# Autodesk Inventor assembly: Quadropod_assembly_v3
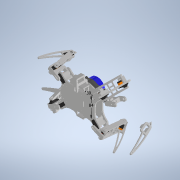
[picture p0: Inventor's stored thumbnail of the model, 180x180]
Saved by Autodesk Inventor 2020.3 (Build 243373000, 373)
## iProperties
Created: 2021-04-02
Part Number: Quadropod_assembly_v3
Document SubType Name: Assembly
Designer: sanyi
Author: sanyi
## Documents named in this file (14)
- C:\Users\sanyi\Documents\Inventor\Quadropod\Quadropod_assembly_v3.iam
- C:\Users\sanyi\Documents\Inventor\Quadropod\BaseBottom_v1.ipt
- C:\Users\sanyi\Documents\Inventor\Quadropod\BaseTop_v1.ipt
- C:\Users\sanyi\Documents\Inventor\Quadropod\LegPin_Middle_v1.ipt
- C:\Users\sanyi\Documents\Inventor\Quadropod\LegPin_Side_v1.ipt
- C:\Users\sanyi\Documents\Inventor\Quadropod\LegPin_Side_v1_MIR.ipt
- C:\Users\sanyi\Documents\Inventor\Quadropod\LegStart_v1.ipt
- C:\Users\sanyi\Documents\Inventor\Quadropod\LegEnd_Right_v2.ipt
- C:\Users\sanyi\Documents\Inventor\Quadropod\LegMiddle_Final_1.ipt
- C:\Users\sanyi\Documents\Inventor\Quadropod\LegPin_v1.ipt
- C:\Users\sanyi\Documents\Inventor\Quadropod\SH-0257MG.ipt
- C:\Users\sanyi\Documents\Inventor\Quadropod\ydlidar x4.ipt
- C:\Users\sanyi\Documents\Inventor\Quadropod\LegEnd_Right_v2_MIR.ipt
- C:\Users\sanyi\Documents\Inventor\Quadropod\LegStart_v1_MIR1.ipt
## Components (44 placed, 13 different names)
1. BaseBottom_v1:1 — Mate:1, Mate:2, Insert:15, Angle:1, Insert:31, Insert:32, Insert:34, Insert:35, Insert:36, Insert:37, Insert:38, Insert:39, Insert:40, Insert:41, Insert:42, Insert:43, Insert:72, Angle:10, Insert:73, Angle:11, Insert:74, Angle:12, Flush:4
2. BaseTop_v1:1 — Insert:75, Insert:76, Insert:77, Insert:78
3. LegPin_Side_v1:1 — Insert:42, Insert:43, Insert:79
4. LegPin_Side_v1_MIR:1 — Insert:40, Insert:41
5. LegPin_Middle_v1:5 — Insert:31, Insert:32, Insert:75
6. LegPin_Middle_v1:2 — Insert:36, Insert:37
7. LegPin_Middle_v1:3 — Insert:38, Insert:39, Insert:76
8. LegPin_Middle_v1:4 — Insert:34, Insert:35
9. LegStart_v1:1 — Insert:16, Insert:17, Angle:2, Flush:2, Insert:29, Insert:30
10. LegEnd_Right_v2:1 — Insert:23, Angle:3, Flush:3, Insert:27, Insert:28
11. LegMiddle_Final_1:1 — Insert:18, Insert:24
12. LegPin_v1:1 — Insert:29, Insert:30
13. LegPin_v1:2 — Insert:27, Insert:28
14. SH-0257MG:1 — Insert:15, Angle:1, Insert:16
15. SH-0257MG:2 — Insert:17, Angle:2, Insert:18
16. SH-0257MG:3 — Insert:23, Angle:3, Insert:24
17. LegStart_v1:2
18. LegEnd_Right_v2:2
19. LegMiddle_Final_1:2
20. LegPin_v1:3
21. LegPin_v1:4
22. SH-0257MG:4 — Insert:72, Angle:10
23. SH-0257MG:5
24. SH-0257MG:6
25. LegStart_v1:3
26. LegEnd_Right_v2:3
27. LegMiddle_Final_1:3
28. LegPin_v1:5
29. LegPin_v1:6
30. SH-0257MG:7 — Insert:73, Angle:11
31. SH-0257MG:8
32. SH-0257MG:9
33. LegStart_v1:4
34. LegEnd_Right_v2:4
35. LegMiddle_Final_1:4
36. LegPin_v1:7
37. LegPin_v1:8
38. SH-0257MG:10 — Insert:74, Angle:12
39. SH-0257MG:11
40. SH-0257MG:12
41. ydlidar x4:1 — Insert:77, Insert:78
42. LegEnd_Right_v2_MIR:1
43. LegStart_v1:5 — Insert:79
44. LegStart_v1_MIR1:1
## Relationships (74: Insert 57, Angle 12, Flush 3, Mate 2)
- Mate:1: BaseBottom_v1:1
- Mate:2: BaseBottom_v1:1
- Insert:15: BaseBottom_v1:1 ↔ SH-0257MG:1
- Angle:1 (0 deg): BaseBottom_v1:1 ↔ SH-0257MG:1
- Insert:16 (0.2 mm): LegStart_v1:1 ↔ SH-0257MG:1
- Insert:17: LegStart_v1:1 ↔ SH-0257MG:2
- Angle:2 (0 deg): LegStart_v1:1 ↔ SH-0257MG:2
- Insert:18 (0.2 mm): LegMiddle_Final_1:1 ↔ SH-0257MG:2
- Insert:23: LegEnd_Right_v2:1 ↔ SH-0257MG:3
- Angle:3 (0 deg): LegEnd_Right_v2:1 ↔ SH-0257MG:3
- Insert:24 (0.2 mm): LegMiddle_Final_1:1 ↔ SH-0257MG:3
- Flush:2 (15.5 mm): LegStart_v1:1
- Flush:3 (14.5 mm): LegEnd_Right_v2:1
- Insert:27: LegEnd_Right_v2:1 ↔ LegPin_v1:2
- Insert:28: LegEnd_Right_v2:1 ↔ LegPin_v1:2
- Insert:29: LegStart_v1:1 ↔ LegPin_v1:1
- Insert:30: LegStart_v1:1 ↔ LegPin_v1:1
- Insert:31: BaseBottom_v1:1 ↔ LegPin_Middle_v1:5
- Insert:32: BaseBottom_v1:1 ↔ LegPin_Middle_v1:5
- Insert:34: BaseBottom_v1:1 ↔ LegPin_Middle_v1:4
- Insert:35: BaseBottom_v1:1 ↔ LegPin_Middle_v1:4
- Insert:36: BaseBottom_v1:1 ↔ LegPin_Middle_v1:2
- Insert:37: BaseBottom_v1:1 ↔ LegPin_Middle_v1:2
- Insert:38: BaseBottom_v1:1 ↔ LegPin_Middle_v1:3
- Insert:39: BaseBottom_v1:1 ↔ LegPin_Middle_v1:3
- Insert:40: BaseBottom_v1:1 ↔ LegPin_Side_v1_MIR:1
- Insert:41: BaseBottom_v1:1 ↔ LegPin_Side_v1_MIR:1
- Insert:42: BaseBottom_v1:1 ↔ LegPin_Side_v1:1
- Insert:43: BaseBottom_v1:1 ↔ LegPin_Side_v1:1
- [Insert] (0.2 mm): LegStart_v1:2 ↔ SH-0257MG:4
- [Insert]: LegStart_v1:2 ↔ SH-0257MG:5
- [Angle] (0 deg): LegStart_v1:2 ↔ SH-0257MG:5
- [Insert] (0.2 mm): LegMiddle_Final_1:2 ↔ SH-0257MG:5
- [Insert]: LegEnd_Right_v2:2 ↔ SH-0257MG:6
- [Angle] (0 deg): LegEnd_Right_v2:2 ↔ SH-0257MG:6
- [Insert] (0.2 mm): LegMiddle_Final_1:2 ↔ SH-0257MG:6
- [Insert]: LegEnd_Right_v2:2 ↔ LegPin_v1:4
- [Insert]: LegEnd_Right_v2:2 ↔ LegPin_v1:4
- [Insert]: LegStart_v1:2 ↔ LegPin_v1:3
- [Insert]: LegStart_v1:2 ↔ LegPin_v1:3
- [Insert] (0.2 mm): LegStart_v1:3 ↔ SH-0257MG:7
- [Insert]: LegStart_v1:3 ↔ SH-0257MG:8
- [Angle] (0 deg): LegStart_v1:3 ↔ SH-0257MG:8
- [Insert] (0.2 mm): LegMiddle_Final_1:3 ↔ SH-0257MG:8
- [Insert]: LegEnd_Right_v2:3 ↔ SH-0257MG:9
- [Angle] (0 deg): LegEnd_Right_v2:3 ↔ SH-0257MG:9
- [Insert] (0.2 mm): LegMiddle_Final_1:3 ↔ SH-0257MG:9
- [Insert]: LegEnd_Right_v2:3 ↔ LegPin_v1:6
- [Insert]: LegEnd_Right_v2:3 ↔ LegPin_v1:6
- [Insert]: LegStart_v1:3 ↔ LegPin_v1:5
- [Insert]: LegStart_v1:3 ↔ LegPin_v1:5
- [Insert] (0.2 mm): LegStart_v1:4 ↔ SH-0257MG:10
- [Insert]: LegStart_v1:4 ↔ SH-0257MG:11
- [Angle] (0 deg): LegStart_v1:4 ↔ SH-0257MG:11
- [Insert] (0.2 mm): LegMiddle_Final_1:4 ↔ SH-0257MG:11
- [Insert]: LegEnd_Right_v2:4 ↔ SH-0257MG:12
- [Angle] (0 deg): LegEnd_Right_v2:4 ↔ SH-0257MG:12
- [Insert] (0.2 mm): LegMiddle_Final_1:4 ↔ SH-0257MG:12
- [Insert]: LegEnd_Right_v2:4 ↔ LegPin_v1:8
- [Insert]: LegEnd_Right_v2:4 ↔ LegPin_v1:8
- [Insert]: LegStart_v1:4 ↔ LegPin_v1:7
- [Insert]: LegStart_v1:4 ↔ LegPin_v1:7
- Insert:72: BaseBottom_v1:1 ↔ SH-0257MG:4
- Angle:10 (0 deg): BaseBottom_v1:1 ↔ SH-0257MG:4
- Insert:73: BaseBottom_v1:1 ↔ SH-0257MG:7
- Angle:11 (0 deg): BaseBottom_v1:1 ↔ SH-0257MG:7
- Insert:74: BaseBottom_v1:1 ↔ SH-0257MG:10
- Angle:12 (0 deg): BaseBottom_v1:1 ↔ SH-0257MG:10
- Flush:4: BaseBottom_v1:1
- Insert:75: BaseTop_v1:1 ↔ LegPin_Middle_v1:5
- Insert:76: BaseTop_v1:1 ↔ LegPin_Middle_v1:3
- Insert:77: BaseTop_v1:1 ↔ ydlidar x4:1
- Insert:78: BaseTop_v1:1 ↔ ydlidar x4:1
- Insert:79 (1 mm): LegPin_Side_v1:1 ↔ LegStart_v1:5
## Named parameters: d60_d40 = 0 mm, d61_d41 = 0 mm, d62_d42 = 0 mm, d63_d43 = 0 mm, d64_d27 = 0 mm, d65_d28 = 0 deg, d66_d29 = 0.2 mm, d67_d19 = 0.2 mm, d68_d20 = 0 mm, d69_d21 = 0 deg, d70_d22 = 0.2 mm, d71_d40 = 0 mm, d72_d41 = 0 mm, d73_d42 = 0 mm, d74_d43 = 0 mm, d75_d27 = 0 mm, d76_d28 = 0 deg, d77_d29 = 0.2 mm, d78_d19 = 0.2 mm, d79_d20 = 0 mm, d80_d21 = 0 deg, d81_d22 = 0.2 mm, d82_d40 = 0 mm, d83_d41 = 0 mm, d84_d42 = 0 mm, d85_d43 = 0 mm, d86_d27 = 0 mm, d87_d28 = 0 deg, d88_d29 = 0.2 mm, d89_d19 = 0.2 mm, d90_d20 = 0 mm, d91_d21 = 0 deg, d92_d22 = 0.2 mm
